# Autodesk Inventor assembly: zlozenie_naped_v2
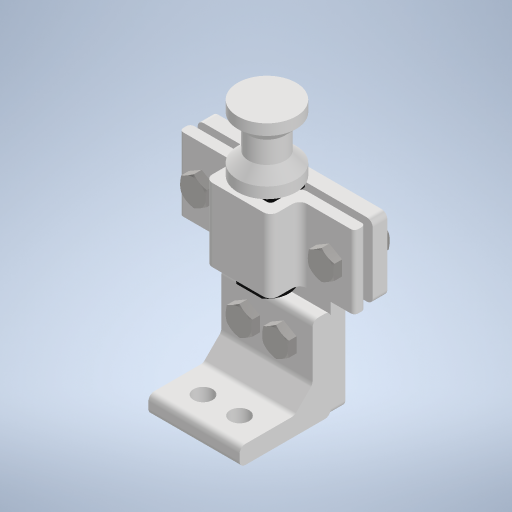
[picture p0: Inventor's stored thumbnail of the model, 512x512]
Saved by Autodesk Inventor 2024.2 (Build 282272000, 272)
## iProperties
Created: 2024-08-27
Part Number: zlozenie_naped_v2
Document SubType Name: Assembly
Designer: Konrad
Author: Konrad
## Documents named in this file (9)
- D:\Inventor\magisterka\prototyp_2\zlozenie_naped_v2.iam
- D:\Inventor\magisterka\prototyp_2\kolo_napedowe.ipt
- D:\Inventor\magisterka\prototyp_2\motor_clamp_v2.ipt
- D:\Inventor\magisterka\prototyp_2\motor_rig_v2.ipt
- D:\Inventor\magisterka\prototyp_2\motor_rig_v3.ipt
- D:\Inventor\grafika3D\dc-motor-GA12-N20.ipt
- C:\Users\Konrad\Documents\Inventor\Content Center Files\R2024\pl-PL\DIN 933\DIN 933 - M4  x 14.ipt
- C:\Users\Konrad\Documents\Inventor\Content Center Files\R2024\pl-PL\DIN 125-1  A\DIN 125 - A 4,3.ipt
- C:\Users\Konrad\Documents\Inventor\Content Center Files\R2024\pl-PL\DIN 934\DIN 934 - M4 x 0,7.ipt
## Components (17 placed, 8 different names)
1. kolo_napedowe:1 — Zestawiające:5, Zestawiające:6, Zestawiające:7
2. motor_clamp_v2:1 — Zestawiające:3, Równoległe:2, Zestawiające:4, Zestawiające:9, Zestawiające:10, Zestawiające:11, Zestawiające:12, Zestawiające:13, Zestawiające:14, Zestawiające:15, Zestawiające:17
3. motor_rig_v2:1 — Zestawiające:1, Zestawiające:2, Równoległe:1, Zestawiające:19, Zestawiające:20, Zestawiające:21, Zestawiające:22, Zestawiające:23, Zestawiające:25
4. motor_rig_v3:1 — Zestawiające:1, Zestawiające:2, Równoległe:1, Zestawiające:8, Zestawiające:9, Zestawiające:10, Zestawiające:16, Zestawiające:18, Zestawiające:24, Zestawiające:26
5. dc-motor-GA12-N20:1 — Zestawiające:3, Równoległe:2, Zestawiające:4, Zestawiające:5, Zestawiające:6, Zestawiające:7, Zestawiające:8
6. DIN 933 - zastąpiona przez DIN EN 24017 M4  x 14:1 — Zestawiające:11, Zestawiające:12
7. DIN 125-1 A A 4,3:1 — Zestawiające:15, Zestawiające:16, Wstawiające:1
8. DIN 934 - zastąpiona przez DIN EN 24032/28673/28674 M4:1 — Wstawiające:1
9. DIN 933 - zastąpiona przez DIN EN 24017 M4  x 14:2 — Zestawiające:13, Zestawiające:14
10. DIN 125-1 A A 4,3:2 — Zestawiające:17, Zestawiające:18, Wstawiające:2
11. DIN 934 - zastąpiona przez DIN EN 24032/28673/28674 M4:2 — Wstawiające:2
12. DIN 933 - zastąpiona przez DIN EN 24017 M4  x 14:3 — Zestawiające:19, Zestawiające:20
13. DIN 125-1 A A 4,3:3 — Zestawiające:23, Zestawiające:24, Wstawiające:3
14. DIN 934 - zastąpiona przez DIN EN 24032/28673/28674 M4:3 — Wstawiające:3
15. DIN 933 - zastąpiona przez DIN EN 24017 M4  x 14:4 — Zestawiające:21, Zestawiające:22
16. DIN 125-1 A A 4,3:4 — Zestawiające:25, Zestawiające:26, Wstawiające:4
17. DIN 934 - zastąpiona przez DIN EN 24032/28673/28674 M4:4 — Wstawiające:4
## Relationships (32: Mate 26, Insert 4, Flush 2)
- Zestawiające:1 [Mate]: motor_rig_v2:1 ↔ motor_rig_v3:1
- Zestawiające:2 [Mate]: motor_rig_v2:1 ↔ motor_rig_v3:1
- Równoległe:1 [Flush]: motor_rig_v2:1 ↔ motor_rig_v3:1
- Zestawiające:3 [Mate]: motor_clamp_v2:1 ↔ dc-motor-GA12-N20:1
- Równoległe:2 [Flush]: motor_clamp_v2:1 ↔ dc-motor-GA12-N20:1
- Zestawiające:4 [Mate]: motor_clamp_v2:1 ↔ dc-motor-GA12-N20:1
- Zestawiające:5 [Mate]: kolo_napedowe:1 ↔ dc-motor-GA12-N20:1
- Zestawiające:6 [Mate]: kolo_napedowe:1 ↔ dc-motor-GA12-N20:1
- Zestawiające:7 [Mate]: kolo_napedowe:1 ↔ dc-motor-GA12-N20:1
- Zestawiające:8 [Mate]: motor_rig_v3:1 ↔ dc-motor-GA12-N20:1
- Zestawiające:9 [Mate]: motor_clamp_v2:1 ↔ motor_rig_v3:1
- Zestawiające:10 [Mate]: motor_clamp_v2:1 ↔ motor_rig_v3:1
- Zestawiające:11 [Mate]: motor_clamp_v2:1 ↔ DIN 933 - zastąpiona przez DIN EN 24017 M4  x 14:1
- Zestawiające:12 [Mate]: motor_clamp_v2:1 ↔ DIN 933 - zastąpiona przez DIN EN 24017 M4  x 14:1
- Zestawiające:13 [Mate]: motor_clamp_v2:1 ↔ DIN 933 - zastąpiona przez DIN EN 24017 M4  x 14:2
- Zestawiające:14 [Mate]: motor_clamp_v2:1 ↔ DIN 933 - zastąpiona przez DIN EN 24017 M4  x 14:2
- Zestawiające:15 [Mate]: motor_clamp_v2:1 ↔ DIN 125-1 A A 4,3:1
- Zestawiające:16 [Mate]: motor_rig_v3:1 ↔ DIN 125-1 A A 4,3:1
- Zestawiające:17 [Mate]: motor_clamp_v2:1 ↔ DIN 125-1 A A 4,3:2
- Zestawiające:18 [Mate]: motor_rig_v3:1 ↔ DIN 125-1 A A 4,3:2
- Wstawiające:1 [Insert]: DIN 125-1 A A 4,3:1 ↔ DIN 934 - zastąpiona przez DIN EN 24032/28673/28674 M4:1
- Wstawiające:2 [Insert]: DIN 125-1 A A 4,3:2 ↔ DIN 934 - zastąpiona przez DIN EN 24032/28673/28674 M4:2
- Zestawiające:19 [Mate]: motor_rig_v2:1 ↔ DIN 933 - zastąpiona przez DIN EN 24017 M4  x 14:3
- Zestawiające:20 [Mate]: motor_rig_v2:1 ↔ DIN 933 - zastąpiona przez DIN EN 24017 M4  x 14:3
- Zestawiające:21 [Mate]: motor_rig_v2:1 ↔ DIN 933 - zastąpiona przez DIN EN 24017 M4  x 14:4
- Zestawiające:22 [Mate]: motor_rig_v2:1 ↔ DIN 933 - zastąpiona przez DIN EN 24017 M4  x 14:4
- Zestawiające:23 [Mate]: motor_rig_v2:1 ↔ DIN 125-1 A A 4,3:3
- Zestawiające:24 [Mate]: motor_rig_v3:1 ↔ DIN 125-1 A A 4,3:3
- Zestawiające:25 [Mate]: motor_rig_v2:1 ↔ DIN 125-1 A A 4,3:4
- Zestawiające:26 [Mate]: motor_rig_v3:1 ↔ DIN 125-1 A A 4,3:4
- Wstawiające:3 [Insert]: DIN 125-1 A A 4,3:3 ↔ DIN 934 - zastąpiona przez DIN EN 24032/28673/28674 M4:3
- Wstawiające:4 [Insert]: DIN 125-1 A A 4,3:4 ↔ DIN 934 - zastąpiona przez DIN EN 24032/28673/28674 M4:4
